# Autodesk Inventor assembly: Iris_On_Carriage
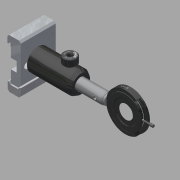
[picture p0: Inventor's stored thumbnail of the model, 180x180]
Saved by Autodesk Inventor 2018 (Build 220112000, 112)
## iProperties
Created: 2018-09-17
Part Number: Iris_On_Carriage
Document SubType Name: Assembly
Designer: Robert Campbell
Author: Robert Campbell
## Documents named in this file (4)
- \\Mac\Home\Dropbox\home\work\Microscopes\SWC_Optics_course_2018\Iris_On_Carriage.iam
- \\Mac\Home\Downloads\LaserAlignment\XT66C4-Step.ipt
- \\Mac\Home\Downloads\LaserAlignment\PH50_M-Solidworks.ipt
- \\Mac\Home\Downloads\LaserAlignment\ID25_M-Solidworks.ipt
## Components (3 placed, 3 different names)
1. XT66C4-Step:1 — Mate:3, Angle:1, Angle:2
2. PH50_M-Solidworks:1 — Mate:1, Mate:2, Mate:3, Angle:1
3. ID25_M-Solidworks:1 — Mate:1, Mate:2, Angle:2
## Relationships (5: Mate 3, Angle 2)
- Mate:1: PH50_M-Solidworks:1 ↔ ID25_M-Solidworks:1
- Mate:2: PH50_M-Solidworks:1 ↔ ID25_M-Solidworks:1
- Mate:3: XT66C4-Step:1 ↔ PH50_M-Solidworks:1
- Angle:1 (0 deg): XT66C4-Step:1 ↔ PH50_M-Solidworks:1
- Angle:2 (0 deg): XT66C4-Step:1 ↔ ID25_M-Solidworks:1
